# Autodesk Inventor assembly: Griper
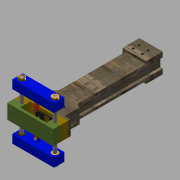
[picture p0: Inventor's stored thumbnail of the model, 180x180]
Saved by Autodesk Inventor 2019 (Build 230136000, 136)
## iProperties
Created: 2021-10-30
Part Number: Griper
Document SubType Name: Assembly
Designer: Mohamed
Author: Mohamed
## Documents named in this file (20)
- F:\Semester 7\Design of mechatronics 1\SSCARA Robot\Griper.iam
- F:\Semester 7\Design of mechatronics 1\SSCARA Robot\g_6mm rod.ipt
- F:\Semester 7\Design of mechatronics 1\SSCARA Robot\g_servo mount 1.ipt
- F:\Semester 7\Design of mechatronics 1\SSCARA Robot\g_servo mount 2.ipt
- F:\Semester 7\Design of mechatronics 1\SSCARA Robot\MG995.ipt
- F:\Semester 7\Design of mechatronics 1\SSCARA Robot\g_servo horn.ipt
- F:\Semester 7\Design of mechatronics 1\SSCARA Robot\g_connector x4.ipt
- F:\Semester 7\Design of mechatronics 1\SSCARA Robot\g_bolt.ipt
- F:\Semester 7\Design of mechatronics 1\SSCARA Robot\g_nut.ipt
- F:\Semester 7\Design of mechatronics 1\SSCARA Robot\g_griper side.ipt
- F:\Semester 7\Design of mechatronics 1\SSCARA Robot\g_griper side2.ipt
- F:\Semester 7\Design of mechatronics 1\SSCARA Robot\g_linear bearing 8mm.ipt
- F:\Semester 7\Design of mechatronics 1\SSCARA Robot\g_mount 1.ipt
- F:\Semester 7\Design of mechatronics 1\SSCARA Robot\g_mount 2.ipt
- F:\Semester 7\Design of mechatronics 1\SSCARA Robot\g_arm1.ipt
- F:\Semester 7\Design of mechatronics 1\SSCARA Robot\g_arm 2.ipt
- F:\Semester 7\Design of mechatronics 1\SSCARA Robot\g_arm3.ipt
- F:\Semester 7\Design of mechatronics 1\SSCARA Robot\g_arm 4.ipt
- F:\Semester 7\Design of mechatronics 1\SSCARA Robot\e_arm holder 1.ipt
- F:\Semester 7\Design of mechatronics 1\SSCARA Robot\e_arm holder 2.ipt
## Components (36 placed, 19 different names)
1. g_6mm rod:1 — Mate:19, Flush:5, Mate:21, Mate:37
2. g_servo mount 1:1 — Mate:1, Mate:2, Mate:3, Flush:4, Mate:19, Flush:5, Mate:20, Flush:6, Mate:32, Flush:11, Flush:12, Mate:38, Mate:39, Mate:40, Mate:41, Mate:42, Mate:43, Mate:49, Mate:51, Mate:52, Mate:58
3. g_servo mount 2:1 — Mate:32, Flush:11, Flush:12
4. MG995:1 — Mate:1, Mate:2, Mate:3, Mate:4, Flush:1, Flush:4
5. g_servo horn:1 — Mate:4, Flush:1, Mate:5, Mate:6, Mate:7, Mate:8, Mate:9, Mate:10, Mate:11, Mate:12, Mate:14, Mate:16
6. g_connector x4:1 — Mate:5, Mate:6, Mate:13, Flush:8
7. g_connector x4:2 — Mate:7, Mate:8, Flush:8, Mate:24, Mate:25, Mate:26, Mate:27
8. g_connector x4:3 — Mate:9, Mate:10, Flush:7, Mate:23, Mate:28, Mate:29
9. g_connector x4:4 — Mate:11, Mate:12, Mate:15, Flush:7
10. g_bolt:1 — Mate:26, Mate:27, Mate:30, Flush:9
11. g_bolt:2 — Mate:15, Mate:16, Mate:18, Flush:3
12. g_bolt:3 — Mate:28, Mate:29, Mate:31, Flush:10
13. g_bolt:4 — Mate:13, Mate:14, Mate:17, Flush:2
14. g_nut:1 — Mate:30, Flush:9
15. g_nut:2 — Mate:31, Flush:10
16. g_nut:3 — Mate:18, Flush:3
17. g_nut:4 — Mate:17, Flush:2
18. g_griper side:1 — Mate:21, Mate:22, Mate:23, Mate:35, Flush:15, Mate:36, Flush:16
19. g_6mm rod:2 — Mate:20, Flush:6, Mate:22
20. g_griper side2:1 — Mate:24, Mate:25, Mate:33, Flush:13, Mate:34, Flush:14
21. g_linear bearing 8mm:1 — Mate:35, Flush:15
22. g_linear bearing 8mm:2 — Mate:33, Flush:13, Mate:37
23. g_linear bearing 8mm:3 — Mate:36, Flush:16
24. g_linear bearing 8mm:4 — Mate:34, Flush:14
25. g_mount 1:1 — Mate:38, Mate:39, Mate:40, Mate:50, Flush:18
26. g_mount 2:1 — Mate:41, Mate:42, Mate:43, Flush:24, Mate:53
27. g_arm 2:2 — Mate:49, Mate:50, Flush:18, Flush:23, Flush:25, Flush:27, Flush:28, Flush:29, Flush:31, Mate:59
28. g_arm3:1 — Flush:26, Mate:54, Mate:55, Flush:27, Flush:28, Flush:29, Flush:30, Mate:56, Mate:57
29. g_arm1:1 — Mate:51, Flush:23, Flush:25, Mate:60, Flush:32, Mate:62
30. g_arm 2:3 — Mate:52, Flush:24, Mate:53
31. g_arm 4:1 — Flush:26, Mate:54, Mate:55
32. g_arm 4:2 — Flush:30, Mate:56, Mate:57
33. g_arm1:2 — Mate:58, Flush:31, Mate:59, Flush:33, Mate:61
34. e_arm holder 1:1 — Mate:60, Flush:32, Flush:33, Flush:34, Flush:35, Flush:36, Flush:37
35. e_arm holder 2:1 — Mate:62, Flush:36, Flush:37
36. e_arm holder 2:2 — Mate:61, Flush:34, Flush:35
## Relationships (89: Mate 57, Flush 32)
- Mate:1 (0.5 mm): g_servo mount 1:1 ↔ MG995:1
- Mate:2 (0.5 mm): g_servo mount 1:1 ↔ MG995:1
- Mate:3: g_servo mount 1:1 ↔ MG995:1
- Mate:4: MG995:1 ↔ g_servo horn:1
- Flush:1 (-0.5 mm): MG995:1 ↔ g_servo horn:1
- Mate:5: g_servo horn:1 ↔ g_connector x4:1
- Mate:6: g_servo horn:1 ↔ g_connector x4:1
- Mate:7: g_servo horn:1 ↔ g_connector x4:2
- Mate:8: g_servo horn:1 ↔ g_connector x4:2
- Mate:9: g_servo horn:1 ↔ g_connector x4:3
- Mate:10: g_servo horn:1 ↔ g_connector x4:3
- Mate:11: g_servo horn:1 ↔ g_connector x4:4
- Mate:12: g_servo horn:1 ↔ g_connector x4:4
- Mate:13: g_connector x4:1 ↔ g_bolt:4
- Mate:14: g_servo horn:1 ↔ g_bolt:4
- Mate:15: g_connector x4:4 ↔ g_bolt:2
- Mate:16: g_servo horn:1 ↔ g_bolt:2
- Mate:17: g_bolt:4 ↔ g_nut:4
- Flush:2: g_bolt:4 ↔ g_nut:4
- Mate:18: g_bolt:2 ↔ g_nut:3
- Flush:3: g_bolt:2 ↔ g_nut:3
- Flush:4 (-1 mm): g_servo mount 1:1 ↔ MG995:1
- Mate:19: g_6mm rod:1 ↔ g_servo mount 1:1
- Flush:5 (-52.5 mm): g_6mm rod:1 ↔ g_servo mount 1:1
- Mate:20: g_servo mount 1:1 ↔ g_6mm rod:2
- Flush:6 (-52.5 mm): g_servo mount 1:1 ↔ g_6mm rod:2
- Mate:21: g_6mm rod:1 ↔ g_griper side:1
- Mate:22: g_griper side:1 ↔ g_6mm rod:2
- Flush:7: g_connector x4:3 ↔ g_connector x4:4
- Flush:8: g_connector x4:1 ↔ g_connector x4:2
- Mate:23: g_connector x4:3 ↔ g_griper side:1
- Mate:24: g_connector x4:2 ↔ g_griper side2:1
- Mate:25: g_connector x4:2 ↔ g_griper side2:1
- Mate:26: g_connector x4:2 ↔ g_bolt:1
- Mate:27: g_connector x4:2 ↔ g_bolt:1
- Mate:28: g_connector x4:3 ↔ g_bolt:3
- Mate:29: g_connector x4:3 ↔ g_bolt:3
- Mate:30: g_bolt:1 ↔ g_nut:1
- Flush:9: g_bolt:1 ↔ g_nut:1
- Mate:31: g_bolt:3 ↔ g_nut:2
- Flush:10: g_bolt:3 ↔ g_nut:2
- Mate:32: g_servo mount 1:1 ↔ g_servo mount 2:1
- Flush:11: g_servo mount 1:1 ↔ g_servo mount 2:1
- Flush:12: g_servo mount 1:1 ↔ g_servo mount 2:1
- Mate:33: g_griper side2:1 ↔ g_linear bearing 8mm:2
- Flush:13: g_griper side2:1 ↔ g_linear bearing 8mm:2
- Mate:34: g_griper side2:1 ↔ g_linear bearing 8mm:4
- Flush:14: g_griper side2:1 ↔ g_linear bearing 8mm:4
- Mate:35: g_griper side:1 ↔ g_linear bearing 8mm:1
- Flush:15: g_griper side:1 ↔ g_linear bearing 8mm:1
- Mate:36: g_griper side:1 ↔ g_linear bearing 8mm:3
- Flush:16: g_griper side:1 ↔ g_linear bearing 8mm:3
- Mate:37: g_6mm rod:1 ↔ g_linear bearing 8mm:2
- Mate:38: g_servo mount 1:1 ↔ g_mount 1:1
- Mate:39: g_servo mount 1:1 ↔ g_mount 1:1
- Mate:40: g_servo mount 1:1 ↔ g_mount 1:1
- Mate:41: g_servo mount 1:1 ↔ g_mount 2:1
- Mate:42: g_servo mount 1:1 ↔ g_mount 2:1
- Mate:43: g_servo mount 1:1 ↔ g_mount 2:1
- Mate:49: g_servo mount 1:1 ↔ g_arm 2:2
- Mate:50: g_mount 1:1 ↔ g_arm 2:2
- Flush:18: g_mount 1:1 ↔ g_arm 2:2
- Mate:51: g_servo mount 1:1 ↔ g_arm1:1
- Flush:23: g_arm 2:2 ↔ g_arm1:1
- Mate:52: g_servo mount 1:1 ↔ g_arm 2:3
- Flush:24: g_mount 2:1 ↔ g_arm 2:3
- Mate:53: g_mount 2:1 ↔ g_arm 2:3
- Flush:25: g_arm 2:2 ↔ g_arm1:1
- Flush:26: g_arm3:1 ↔ g_arm 4:1
- Mate:54: g_arm3:1 ↔ g_arm 4:1
- Mate:55: g_arm3:1 ↔ g_arm 4:1
- Flush:27: g_arm 2:2 ↔ g_arm3:1
- Flush:28: g_arm 2:2 ↔ g_arm3:1
- Flush:29: g_arm 2:2 ↔ g_arm3:1
- Flush:30: g_arm3:1 ↔ g_arm 4:2
- Mate:56: g_arm3:1 ↔ g_arm 4:2
- Mate:57: g_arm3:1 ↔ g_arm 4:2
- Mate:58: g_servo mount 1:1 ↔ g_arm1:2
- Flush:31: g_arm 2:2 ↔ g_arm1:2
- Mate:59: g_arm 2:2 ↔ g_arm1:2
- Mate:60: g_arm1:1 ↔ e_arm holder 1:1
- Flush:32: g_arm1:1 ↔ e_arm holder 1:1
- Flush:33: g_arm1:2 ↔ e_arm holder 1:1
- Mate:61: g_arm1:2 ↔ e_arm holder 2:2
- Flush:34: e_arm holder 1:1 ↔ e_arm holder 2:2
- Flush:35: e_arm holder 1:1 ↔ e_arm holder 2:2
- Mate:62: g_arm1:1 ↔ e_arm holder 2:1
- Flush:36: e_arm holder 1:1 ↔ e_arm holder 2:1
- Flush:37: e_arm holder 1:1 ↔ e_arm holder 2:1
